# Autodesk Inventor assembly: Assembly1
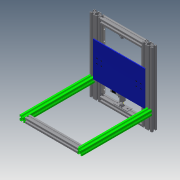
[picture p0: Inventor's stored thumbnail of the model, 180x180]
Saved by Autodesk Inventor 2016 (Build 200138000, 138)
## iProperties
Created: 2017-05-10
Part Number: Assembly1
Document SubType Name: Assembly
Designer: Spark Electronics
Author: Spark Electronics
## Documents named in this file (15)
- C:\Users\Owner\Documents\REZ_RAP\Assembly1.iam
- C:\Users\Owner\Documents\REZ_RAP\Y_CARRIAGE.ipt
- C:\Users\Owner\Documents\REZ_RAP\Y_carriage_90_bearing_mount.ipt
- C:\Users\Owner\Documents\REZ_RAP\15mm_bearing_rail_carriage.ipt
- C:\Users\Owner\Documents\REZ_RAP\y_Carriage_flat_head_8mm.ipt
- C:\Users\Owner\Documents\REZ_RAP\Y_carriage_bearing_rail.ipt
- C:\Users\Owner\Documents\REZ_RAP\ALuminum_extrusion_short.ipt
- C:\Users\Owner\Documents\REZ_RAP\Aluminum_extrusion_Z.ipt
- C:\Users\Owner\Documents\REZ_RAP\Aluminum_extrusion_Z_top.ipt
- C:\Users\Owner\Documents\REZ_RAP\Aluminum_extrusion_60_wide.ipt
- C:\Users\Owner\Documents\REZ_RAP\Nema 17.iam
- C:\Users\Owner\Documents\REZ_RAP\y_motor.ipt
- C:\Users\Owner\Documents\REZ_RAP\bearing_y_carriage.ipt
- C:\Users\Owner\Documents\REZ_RAP\y_idle.ipt
- C:\Users\Owner\Documents\REZ_RAP\rack.ipt
## Components (28 placed, 14 different names)
1. Y_CARRIAGE:1 — Mate:9, Mate:10, Mate:57, Flush:42, Flush:43
2. y_Carriage_flat_head_8mm:1
3. y_Carriage_flat_head_8mm:2
4. y_Carriage_flat_head_8mm:3
5. y_Carriage_flat_head_8mm:4
6. y_Carriage_flat_head_8mm:5
7. y_Carriage_flat_head_8mm:6
8. y_Carriage_flat_head_8mm:7
9. y_Carriage_flat_head_8mm:8
10. Y_carriage_90_bearing_mount:1 — Mate:9, Mate:12, Mate:15, Mate:16
11. Y_carriage_90_bearing_mount:2 — Mate:10, Mate:11, Mate:13, Mate:14
12. 15mm_bearing_rail_carriage:1 — Mate:12, Mate:15, Mate:16, Mate:20, Mate:22, Mate:25, Mate:26
13. 15mm_bearing_rail_carriage:2 — Mate:11, Mate:13, Mate:14, Mate:19, Mate:21, Mate:23, Mate:24
14. Y_carriage_bearing_rail:1 — Mate:19, Mate:21, Mate:23, Mate:24, Flush:11, Mate:30
15. Y_carriage_bearing_rail:2 — Mate:20, Mate:22, Mate:25, Mate:26, Flush:11, Mate:31, Mate:32, Flush:24
16. Aluminum_extrusion_60_wide:1 — Mate:31, Flush:24, Flush:31, Flush:32, Mate:39, Mate:41, Flush:34, Flush:35, Mate:43, Flush:37
17. Aluminum_extrusion_60_wide:2 — Mate:30, Flush:31, Flush:32, Mate:40, Flush:33, Flush:36, Mate:42
18. ALuminum_extrusion_short:1 — Mate:32, Mate:41, Flush:34, Flush:35, Flush:40, Mate:46
19. ALuminum_extrusion_short:2 — Mate:39, Mate:40, Flush:33, Mate:54, Flush:41
20. Aluminum_extrusion_Z:1 — Flush:36, Mate:42, Flush:38
21. Aluminum_extrusion_Z:2 — Mate:38, Flush:29, Flush:30, Mate:43, Flush:37
22. Aluminum_extrusion_Z_top:1 — Mate:38, Flush:29, Flush:30, Flush:38
23. Nema 17:1 [sub-assembly] — Mate:47, Mate:48, Mate:49, Mate:50, Mate:51, Mate:52, Mate:53
24. y_motor:1 — Mate:44, Mate:45, Flush:40, Mate:46, Mate:47, Mate:48, Mate:49, Mate:50, Mate:51, Mate:52, Mate:53
25. bearing_y_carriage:1 — Mate:44, Mate:45
26. y_idle:1 — Mate:54, Flush:41, Mate:55, Mate:56
27. bearing_y_carriage:2 — Mate:55, Mate:56
28. rack:1 — Mate:57, Flush:42, Flush:43
## Relationships (90: Mate 54, Flush 36)
- [Mate]: Y_CARRIAGE:1 ↔ y_Carriage_flat_head_8mm:1
- [Mate]: Y_CARRIAGE:1 ↔ y_Carriage_flat_head_8mm:2
- [Mate]: Y_CARRIAGE:1 ↔ y_Carriage_flat_head_8mm:3
- [Mate]: Y_CARRIAGE:1 ↔ y_Carriage_flat_head_8mm:4
- [Mate]: Y_CARRIAGE:1 ↔ y_Carriage_flat_head_8mm:8
- [Mate]: Y_CARRIAGE:1 ↔ y_Carriage_flat_head_8mm:7
- [Mate]: Y_CARRIAGE:1 ↔ y_Carriage_flat_head_8mm:5
- [Mate]: Y_CARRIAGE:1 ↔ y_Carriage_flat_head_8mm:6
- [Flush]: Y_CARRIAGE:1 ↔ y_Carriage_flat_head_8mm:1
- [Flush]: Y_CARRIAGE:1 ↔ y_Carriage_flat_head_8mm:2
- [Flush]: Y_CARRIAGE:1 ↔ y_Carriage_flat_head_8mm:3
- [Flush]: Y_CARRIAGE:1 ↔ y_Carriage_flat_head_8mm:4
- [Flush]: Y_CARRIAGE:1 ↔ y_Carriage_flat_head_8mm:6
- [Flush]: Y_CARRIAGE:1 ↔ y_Carriage_flat_head_8mm:5
- [Flush]: Y_CARRIAGE:1 ↔ y_Carriage_flat_head_8mm:8
- [Flush]: Y_CARRIAGE:1 ↔ y_Carriage_flat_head_8mm:7
- Mate:9: Y_CARRIAGE:1 ↔ Y_carriage_90_bearing_mount:1
- Mate:10: Y_CARRIAGE:1 ↔ Y_carriage_90_bearing_mount:2
- Mate:11: Y_carriage_90_bearing_mount:2 ↔ 15mm_bearing_rail_carriage:2
- Mate:12: Y_carriage_90_bearing_mount:1 ↔ 15mm_bearing_rail_carriage:1
- Mate:13: Y_carriage_90_bearing_mount:2 ↔ 15mm_bearing_rail_carriage:2
- Mate:14: Y_carriage_90_bearing_mount:2 ↔ 15mm_bearing_rail_carriage:2
- Mate:15: Y_carriage_90_bearing_mount:1 ↔ 15mm_bearing_rail_carriage:1
- Mate:16: Y_carriage_90_bearing_mount:1 ↔ 15mm_bearing_rail_carriage:1
- [Mate]: y_Carriage_flat_head_8mm:5 ↔ Y_carriage_90_bearing_mount:2
- [Mate]: y_Carriage_flat_head_8mm:1 ↔ Y_carriage_90_bearing_mount:1
- Mate:19: 15mm_bearing_rail_carriage:2 ↔ Y_carriage_bearing_rail:1
- Mate:20: 15mm_bearing_rail_carriage:1 ↔ Y_carriage_bearing_rail:2
- Mate:21: 15mm_bearing_rail_carriage:2 ↔ Y_carriage_bearing_rail:1
- Mate:22: 15mm_bearing_rail_carriage:1 ↔ Y_carriage_bearing_rail:2
- Mate:23: 15mm_bearing_rail_carriage:2 ↔ Y_carriage_bearing_rail:1
- Mate:24: 15mm_bearing_rail_carriage:2 ↔ Y_carriage_bearing_rail:1
- Mate:25: 15mm_bearing_rail_carriage:1 ↔ Y_carriage_bearing_rail:2
- Mate:26: 15mm_bearing_rail_carriage:1 ↔ Y_carriage_bearing_rail:2
- Flush:11: Y_carriage_bearing_rail:1 ↔ Y_carriage_bearing_rail:2
- [Flush]: Aluminum_extrusion_60_wide:2 ↔ ALuminum_extrusion_short:1
- [Flush]: Aluminum_extrusion_60_wide:1 ↔ ALuminum_extrusion_short:1
- [Flush]: Aluminum_extrusion_60_wide:1 ↔ ALuminum_extrusion_short:1
- [Flush]: Aluminum_extrusion_60_wide:2 ↔ ALuminum_extrusion_short:1
- [Flush]: Aluminum_extrusion_60_wide:1 ↔ ALuminum_extrusion_short:1
- [Flush]: Aluminum_extrusion_60_wide:1 ↔ ALuminum_extrusion_short:2
- [Flush]: Aluminum_extrusion_60_wide:2 ↔ ALuminum_extrusion_short:2
- [Flush]: Aluminum_extrusion_60_wide:2 ↔ ALuminum_extrusion_short:2
- Mate:30 (-4 mm): Y_carriage_bearing_rail:1 ↔ Aluminum_extrusion_60_wide:2
- Mate:31 (-4 mm): Y_carriage_bearing_rail:2 ↔ Aluminum_extrusion_60_wide:1
- Mate:32 (12.7 mm): Y_carriage_bearing_rail:2 ↔ ALuminum_extrusion_short:1
- Flush:24 (-7.62 mm): Y_carriage_bearing_rail:2 ↔ Aluminum_extrusion_60_wide:1
- [Mate]: Aluminum_extrusion_60_wide:1 ↔ ALuminum_extrusion_short:1
- [Mate]: Aluminum_extrusion_60_wide:2 ↔ ALuminum_extrusion_short:1
- [Mate]: Aluminum_extrusion_60_wide:1 ↔ ALuminum_extrusion_short:2
- [Flush] (228.6 mm): Aluminum_extrusion_60_wide:2 ↔ Aluminum_extrusion_Z:1
- [Flush] (228.6 mm): Aluminum_extrusion_60_wide:1 ↔ Aluminum_extrusion_Z:2
- [Mate] (3 mm): Aluminum_extrusion_60_wide:2 ↔ Aluminum_extrusion_Z:1
- [Mate] (3 mm): Aluminum_extrusion_60_wide:1 ↔ Aluminum_extrusion_Z:2
- [Flush] (-38.1 mm): Aluminum_extrusion_60_wide:1 ↔ Aluminum_extrusion_Z:2
- [Flush] (-38.1 mm): Aluminum_extrusion_60_wide:2 ↔ Aluminum_extrusion_Z:1
- Mate:38: Aluminum_extrusion_Z:2 ↔ Aluminum_extrusion_Z_top:1
- Flush:29: Aluminum_extrusion_Z:2 ↔ Aluminum_extrusion_Z_top:1
- Flush:30: Aluminum_extrusion_Z:2 ↔ Aluminum_extrusion_Z_top:1
- Flush:31: Aluminum_extrusion_60_wide:1 ↔ Aluminum_extrusion_60_wide:2
- Flush:32: Aluminum_extrusion_60_wide:1 ↔ Aluminum_extrusion_60_wide:2
- Mate:39: Aluminum_extrusion_60_wide:1 ↔ ALuminum_extrusion_short:2
- Mate:40: Aluminum_extrusion_60_wide:2 ↔ ALuminum_extrusion_short:2
- Flush:33: Aluminum_extrusion_60_wide:2 ↔ ALuminum_extrusion_short:2
- Mate:41: Aluminum_extrusion_60_wide:1 ↔ ALuminum_extrusion_short:1
- Flush:34: Aluminum_extrusion_60_wide:1 ↔ ALuminum_extrusion_short:1
- Flush:35: Aluminum_extrusion_60_wide:1 ↔ ALuminum_extrusion_short:1
- Flush:36: Aluminum_extrusion_60_wide:2 ↔ Aluminum_extrusion_Z:1
- Mate:42: Aluminum_extrusion_60_wide:2 ↔ Aluminum_extrusion_Z:1
- Mate:43: Aluminum_extrusion_60_wide:1 ↔ Aluminum_extrusion_Z:2
- Flush:37: Aluminum_extrusion_60_wide:1 ↔ Aluminum_extrusion_Z:2
- Flush:38: Aluminum_extrusion_Z:1 ↔ Aluminum_extrusion_Z_top:1
- Mate:44: y_motor:1 ↔ bearing_y_carriage:1
- Mate:45 (0.127 mm): y_motor:1 ↔ bearing_y_carriage:1
- Flush:40: ALuminum_extrusion_short:1 ↔ y_motor:1
- Mate:46: ALuminum_extrusion_short:1 ↔ y_motor:1
- Mate:47: Nema 17:1 ↔ y_motor:1
- Mate:48: Nema 17:1 ↔ y_motor:1
- Mate:49: Nema 17:1 ↔ y_motor:1
- Mate:50: Nema 17:1 ↔ y_motor:1
- Mate:51: Nema 17:1 ↔ y_motor:1
- Mate:52: Nema 17:1 ↔ y_motor:1
- Mate:53: Nema 17:1 ↔ y_motor:1
- Mate:54: ALuminum_extrusion_short:2 ↔ y_idle:1
- Flush:41 (5.08 mm): ALuminum_extrusion_short:2 ↔ y_idle:1
- Mate:55: y_idle:1 ↔ bearing_y_carriage:2
- Mate:56 (0.127 mm): y_idle:1 ↔ bearing_y_carriage:2
- Mate:57: Y_CARRIAGE:1 ↔ rack:1
- Flush:42 (152.4 mm): Y_CARRIAGE:1 ↔ rack:1
- Flush:43: Y_CARRIAGE:1 ↔ rack:1
